# Autodesk Inventor assembly: passive encoder
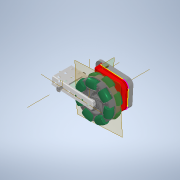
[picture p0: Inventor's stored thumbnail of the model, 180x180]
Saved by Autodesk Inventor 2020 (Build 240168000, 168)
## iProperties
Created: 2020-04-30
Part Number: passive encoder
Document SubType Name: Assembly
Designer: sophi
Author: sophi
## Documents named in this file (10)
- C:\Users\sophi\School\VEX-90819-2021\Inventor Files\Assemblies\passive encoder.iam
- C:\Users\sophi\School\VEX-90819-2021\Inventor Files\Motion\2.75 inch Omni-Directional Wheel.iam
- C:\Users\sophi\School\VEX-90819-2021\Inventor Files\Structure\C-Channel\C-Channel 1x3x1x10 Hole Cut.ipt
- C:\Users\sophi\School\VEX-90819-2021\Inventor Files\Sensors\Optical Shaft Encoder.iam
- C:\Users\sophi\School\VEX-90819-2021\Inventor Files\Motion\Shafts and Related\Shaft 3 inch.ipt
- C:\Users\sophi\School\VEX-90819-2021\Inventor Files\Motion\Shafts and Related\Nylon Spacer 0.125 inch.ipt
- C:\Users\sophi\School\VEX-90819-2021\Inventor Files\Motion\Shafts and Related\Shaft Collar.iam
- C:\Users\sophi\School\VEX-90819-2021\Inventor Files\Structure\Screws and Nuts\Star Screw 8-32 x 2 inches long.ipt
- C:\Users\sophi\School\VEX-90819-2021\Inventor Files\Structure\Screws and Nuts\Nut 8-32 Nylock.ipt
- C:\Users\sophi\School\VEX-90819-2021\Inventor Files\Structure\Screws and Nuts\Star Screw 8-32 x 1 inch long.ipt
## Components (11 placed, 9 different names)
1. 2.75 inch Omni-Directional Wheel:1 [sub-assembly] — Mate:8, Mate:9, Angle:2, Mate:21, Angle:5, Mate:25
2. C-Channel 1x3x1x10 Hole Cut:1 — Mate:1, Mate:2, Mate:3, Mate:4, Angle:1, Mate:14, Mate:15, Mate:16, Mate:17, Angle:4, Mate:23, Mate:24, Mate:26, Mate:27, Mate:28, Flush:1, Mate:32, Mate:33, Mate:34, Mate:35, Angle:6, Mate:40, Mate:42, Mate:44
3. Optical Shaft Encoder:1 [sub-assembly] — Mate:9, Mate:11, Angle:3, Mate:20, Angle:4, Insert:1, Mate:31
4. Shaft 3 inch:1 — Mate:10, Angle:2, Angle:3, Flush:1
5. Nylon Spacer 0.125 inch:1 — Insert:1
6. Shaft Collar:1 [sub-assembly] — Mate:21, Mate:22, Mate:23
7. Shaft Collar:2 [sub-assembly] — Mate:22, Mate:24, Mate:30
8. Star Screw 8-32 x 2 inches long:1 — Mate:39, Mate:40, Mate:41
9. Shaft Collar:3 [sub-assembly] — Mate:30, Mate:31
10. Nut 8-32 Nylock:1 — Mate:41, Mate:42
11. Star Screw 8-32 x 1 inch long:1 — Mate:43, Mate:44
## Relationships (52: Mate 44, Angle 6, Insert 1, Flush 1)
- Mate:1: C-Channel 1x3x1x10 Hole Cut:1
- Mate:2: C-Channel 1x3x1x10 Hole Cut:1
- Mate:3: C-Channel 1x3x1x10 Hole Cut:1
- Mate:4: C-Channel 1x3x1x10 Hole Cut:1
- Mate:5
- Mate:6
- Mate:7
- Angle:1 (0 deg): C-Channel 1x3x1x10 Hole Cut:1
- Mate:8: 2.75 inch Omni-Directional Wheel:1
- Mate:9: 2.75 inch Omni-Directional Wheel:1 ↔ Optical Shaft Encoder:1
- Mate:10: Shaft 3 inch:1
- Mate:11: Optical Shaft Encoder:1
- Angle:2 (0 deg): 2.75 inch Omni-Directional Wheel:1 ↔ Shaft 3 inch:1
- Angle:3 (0 deg): Optical Shaft Encoder:1 ↔ Shaft 3 inch:1
- [Mate]: Nylon Spacer 0.125 inch:1
- [Mate]: C-Channel 1x3x1x10 Hole Cut:1 ↔ Nylon Spacer 0.125 inch:1
- Mate:14: C-Channel 1x3x1x10 Hole Cut:1
- Mate:15: C-Channel 1x3x1x10 Hole Cut:1
- Mate:16: C-Channel 1x3x1x10 Hole Cut:1
- Mate:17: C-Channel 1x3x1x10 Hole Cut:1
- Mate:18
- Mate:19
- Mate:20: Optical Shaft Encoder:1
- Angle:4 (0 deg): C-Channel 1x3x1x10 Hole Cut:1 ↔ Optical Shaft Encoder:1
- Insert:1: Optical Shaft Encoder:1 ↔ Nylon Spacer 0.125 inch:1
- Mate:21: 2.75 inch Omni-Directional Wheel:1 ↔ Shaft Collar:1
- Mate:22: Shaft Collar:1 ↔ Shaft Collar:2
- Mate:23: C-Channel 1x3x1x10 Hole Cut:1 ↔ Shaft Collar:1
- Mate:24: C-Channel 1x3x1x10 Hole Cut:1 ↔ Shaft Collar:2
- Angle:5 (0 deg): 2.75 inch Omni-Directional Wheel:1
- Mate:25: 2.75 inch Omni-Directional Wheel:1
- Mate:26: C-Channel 1x3x1x10 Hole Cut:1
- Mate:27: C-Channel 1x3x1x10 Hole Cut:1
- Mate:28: C-Channel 1x3x1x10 Hole Cut:1
- Mate:29
- Mate:30: Shaft Collar:2 ↔ Shaft Collar:3
- Mate:31: Optical Shaft Encoder:1 ↔ Shaft Collar:3
- Flush:1 (2.54 mm): C-Channel 1x3x1x10 Hole Cut:1 ↔ Shaft 3 inch:1
- Mate:32: C-Channel 1x3x1x10 Hole Cut:1
- Mate:33: C-Channel 1x3x1x10 Hole Cut:1
- Mate:34: C-Channel 1x3x1x10 Hole Cut:1
- Mate:35: C-Channel 1x3x1x10 Hole Cut:1
- Mate:36
- Mate:37
- Mate:38
- Angle:6 (0 deg): C-Channel 1x3x1x10 Hole Cut:1
- Mate:39: Star Screw 8-32 x 2 inches long:1
- Mate:40 (6.35 mm): C-Channel 1x3x1x10 Hole Cut:1 ↔ Star Screw 8-32 x 2 inches long:1
- Mate:41: Star Screw 8-32 x 2 inches long:1 ↔ Nut 8-32 Nylock:1
- Mate:42: C-Channel 1x3x1x10 Hole Cut:1 ↔ Nut 8-32 Nylock:1
- Mate:43: Star Screw 8-32 x 1 inch long:1
- Mate:44: C-Channel 1x3x1x10 Hole Cut:1 ↔ Star Screw 8-32 x 1 inch long:1
